# Autodesk Inventor assembly: Ensamblaje3
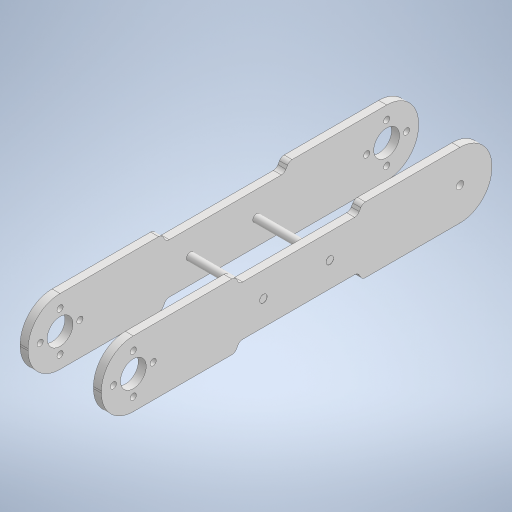
[picture p0: Inventor's stored thumbnail of the model, 512x512]
Saved by Autodesk Inventor 2023 (Build 270158000, 158)
## iProperties
Created: 2024-10-09
Part Number: Ensamblaje3
Document SubType Name: Assembly
Designer: sebas
Author: sebas
## Documents named in this file (2)
- C:\Users\sebas\OneDrive\Documentos\ILLERO_MODELADO_ROBOT\Ensamblaje3.iam
- C:\Users\sebas\OneDrive\Documentos\ILLERO_MODELADO_ROBOT\Pieza_eslabon_3.ipt
## Components (1 placed, 1 different names)
1. Pieza_eslabon_3:1 — Coincidencia:1, Coincidencia:2
## Relationships (2: Mate 2)
- Coincidencia:1 [Mate]: Pieza_eslabon_3:1
- Coincidencia:2 [Mate]: Pieza_eslabon_3:1
